# Autodesk Inventor assembly: Team_2374
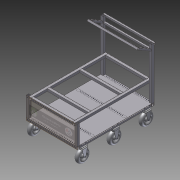
[picture p0: Inventor's stored thumbnail of the model, 180x180]
Saved by Autodesk Inventor 2012 (Build 160160000, 160)
## iProperties
Created: 2011-10-19
Part Number: Team_2374
Document SubType Name: Assembly
Designer: Ian Walters
Mass: 25411.4 g
Surface Area: 59424.9 cm^2
Volume: 9376.89 cm^3
Density: 2.71 g/cm^3
_SolveAssemblyDoc: Frame Generator Solve Assembly
_Version: 15.0.0
Author: Ian Walters
## Documents named in this file (32)
- C:\Users\robotics\Dropbox\CAD Inventor\Preseason Projects\Cart Competition Cart\Team 2374\Team_2374.iam
- C:\Users\robotics\Dropbox\CAD Inventor\Preseason Projects\Cart Competition Cart\Team 2374\Cart Skeleton.ipt
- C:\Users\robotics\Dropbox\CAD Inventor\Preseason Projects\Cart Competition Cart\Team 2374\Team_2374\Frame\Cart Frame.iam
- C:\Users\robotics\Dropbox\CAD Inventor\Preseason Projects\Cart Competition Cart\Team 2374\Bottom Sheet.ipt
- C:\Users\robotics\Dropbox\CAD Inventor\Preseason Projects\Cart Competition Cart\Team 2374\IFI 114 - .1875 x 0.25.ipt
- C:\Users\robotics\Dropbox\CAD Inventor\Preseason Projects\Cart Competition Cart\Team 2374\Fixed Caster.iam
- C:\Users\robotics\Dropbox\CAD Inventor\Preseason Projects\Cart Competition Cart\Team 2374\Team_2374\Design Accelerator\Bolted Connection1.iam
- C:\Users\robotics\Dropbox\CAD Inventor\Preseason Projects\Cart Competition Cart\Team 2374\Team_2374\Design Accelerator\Bolted Connection2.iam
- C:\Users\robotics\Dropbox\CAD Inventor\Preseason Projects\Cart Competition Cart\Team 2374\Team_2374\Design Accelerator\Bolted Connection3.iam
- C:\Users\robotics\Dropbox\CAD Inventor\Preseason Projects\Cart Competition Cart\Team 2374\Team_2374\Design Accelerator\Bolted Connection4.iam
- C:\Users\robotics\Dropbox\CAD Inventor\Preseason Projects\Cart Competition Cart\Team 2374\Team_2374\Design Accelerator\Bolted Connection5.iam
- C:\Users\robotics\Dropbox\CAD Inventor\Preseason Projects\Cart Competition Cart\Team 2374\Team_2374\Design Accelerator\Bolted Connection6.iam
- C:\Users\robotics\Dropbox\CAD Inventor\Preseason Projects\Cart Competition Cart\Team 2374\Team_2374\Design Accelerator\Bolted Connection7.iam
- C:\Users\robotics\Dropbox\CAD Inventor\Preseason Projects\Cart Competition Cart\Team 2374\Team_2374\Design Accelerator\Bolted Connection8.iam
- C:\Users\robotics\Dropbox\CAD Inventor\Preseason Projects\Cart Competition Cart\Team 2374\Front Screen.ipt
- C:\Users\robotics\Dropbox\CAD Inventor\Preseason Projects\Cart Competition Cart\Team 2374\Rotation Caster.iam
- C:\Users\robotics\Dropbox\CAD Inventor\Preseason Projects\Cart Competition Cart\Team 2374\Team_2374\Design Accelerator\Bolted Connection9.iam
- C:\Users\robotics\Dropbox\CAD Inventor\Preseason Projects\Cart Competition Cart\Team 2374\Team_2374\Design Accelerator\Bolted Connection10.iam
- C:\Users\robotics\Dropbox\CAD Inventor\Preseason Projects\Cart Competition Cart\Team 2374\Team_2374\Design Accelerator\Bolted Connection11.iam
- C:\Users\robotics\Dropbox\CAD Inventor\Preseason Projects\Cart Competition Cart\Team 2374\Team_2374\Design Accelerator\Bolted Connection12.iam
- C:\Users\robotics\Dropbox\CAD Inventor\Preseason Projects\Cart Competition Cart\Team 2374\Team_2374\Design Accelerator\Bolted Connection13.iam
- C:\Users\robotics\Dropbox\CAD Inventor\Preseason Projects\Cart Competition Cart\Team 2374\Team_2374\Design Accelerator\Bolted Connection14.iam
- C:\Users\robotics\Dropbox\CAD Inventor\Preseason Projects\Cart Competition Cart\Team 2374\Team_2374\Design Accelerator\Bolted Connection15.iam
- C:\Users\robotics\Dropbox\CAD Inventor\Preseason Projects\Cart Competition Cart\Team 2374\Team_2374\Design Accelerator\Bolted Connection16.iam
- C:\Users\robotics\Dropbox\CAD Inventor\Preseason Projects\Cart Competition Cart\Team 2374\Team_2374\Design Accelerator\Bolted Connection17.iam
- C:\Users\robotics\Dropbox\CAD Inventor\Preseason Projects\Cart Competition Cart\Team 2374\Team_2374\Design Accelerator\Bolted Connection18.iam
- C:\Users\robotics\Dropbox\CAD Inventor\Preseason Projects\Cart Competition Cart\Team 2374\Team_2374\Design Accelerator\Bolted Connection19.iam
- C:\Users\robotics\Dropbox\CAD Inventor\Preseason Projects\Cart Competition Cart\Team 2374\Team_2374\Design Accelerator\Bolted Connection20.iam
- C:\Users\robotics\Dropbox\CAD Inventor\Preseason Projects\Cart Competition Cart\Team 2374\Team_2374\Design Accelerator\Bolted Connection21.iam
- C:\Users\robotics\Dropbox\CAD Inventor\Preseason Projects\Cart Competition Cart\Team 2374\Team_2374\Design Accelerator\Bolted Connection22.iam
- C:\Users\robotics\Dropbox\CAD Inventor\Preseason Projects\Cart Competition Cart\Team 2374\Team_2374\Design Accelerator\Bolted Connection23.iam
- C:\Users\robotics\Dropbox\CAD Inventor\Preseason Projects\Cart Competition Cart\Team 2374\Team_2374\Design Accelerator\Bolted Connection24.iam
## Components (200 placed, 8 different names)
1. Cart Skeleton:1
2. Cart Frame:1 [sub-assembly] — Mate:1, Mate:2, Mate:3, Mate:4, Mate:5, Flush:1, Flush:2, Mate:26, Insert:11, Insert:12, Mate:29, Mate:30, Mate:31, Mate:32, Mate:33, Mate:34, Mate:35, Mate:36, Mate:37, Mate:38, Mate:39, Mate:40, Mate:41, Mate:42, Mate:43, Mate:44, Mate:45, Insert:13, Mate:46, Insert:14, Mate:47, Insert:15, Mate:48, Insert:16, Mate:49, Mate:50, Mate:51, Mate:52, Mate:53, Mate:54, Mate:55, Mate:56, Mate:57, Mate:58, Mate:59, Mate:60, Mate:61, Mate:62, Mate:63, Mate:64, Mate:65, Mate:66, Mate:67, Mate:68, Mate:69, Mate:70, Mate:71, Mate:72, Mate:73, Mate:74, Mate:75, Mate:76, Mate:77, Mate:78, Mate:79, Mate:80
3. Bottom Sheet:1 — Mate:1, Mate:2, Mate:3, Insert:1, Insert:2, Insert:3, Insert:4
4. Fixed Caster:1 [sub-assembly] — Mate:5, Insert:11
5. Fixed Caster:2 [sub-assembly] — Mate:4, Insert:12
6. Bolted Connection:1 [sub-assembly] — Mate:43, Mate:44
7. Bolted Connection:2 [sub-assembly] — Mate:29, Mate:30
8. Bolted Connection:3 [sub-assembly] — Mate:31, Mate:32
9. Bolted Connection:4 [sub-assembly] — Mate:33, Mate:34
10. Bolted Connection:5 [sub-assembly] — Mate:35, Mate:36
11. Bolted Connection:6 [sub-assembly] — Mate:37, Mate:38
12. Bolted Connection:7 [sub-assembly] — Mate:39, Mate:40
13. Bolted Connection:8 [sub-assembly] — Mate:41, Mate:42
14. Front Screen:1 — Flush:1, Flush:2, Mate:26, Insert:7, Insert:8, Insert:9, Insert:10
15. IFI 114 - .1875 x 0.25:109 — Insert:7
16. IFI 114 - .1875 x 0.25:142 — Insert:10
17. Rotation Caster:1 [sub-assembly] — Mate:45, Insert:13
18. Rotation Caster:2 [sub-assembly] — Mate:46, Insert:14
19. Rotation Caster:3 [sub-assembly] — Mate:47, Insert:15
20. Rotation Caster:4 [sub-assembly] — Mate:48, Insert:16
21. Bolted Connection:9 [sub-assembly] — Mate:49, Mate:50
22. Bolted Connection:10 [sub-assembly] — Mate:51, Mate:52
23. Bolted Connection:11 [sub-assembly] — Mate:53, Mate:54
24. Bolted Connection:12 [sub-assembly] — Mate:55, Mate:56
25. Bolted Connection:13 [sub-assembly] — Mate:57, Mate:58
26. Bolted Connection:14 [sub-assembly] — Mate:59, Mate:60
27. Bolted Connection:15 [sub-assembly] — Mate:61, Mate:62
28. Bolted Connection:16 [sub-assembly] — Mate:63, Mate:64
29. Bolted Connection:17 [sub-assembly] — Mate:65, Mate:66
30. Bolted Connection:18 [sub-assembly] — Mate:67, Mate:68
31. Bolted Connection:19 [sub-assembly] — Mate:69, Mate:70
32. Bolted Connection:20 [sub-assembly] — Mate:71, Mate:72
33. Bolted Connection:21 [sub-assembly] — Mate:73, Mate:74
34. Bolted Connection:22 [sub-assembly] — Mate:75, Mate:76
35. Bolted Connection:23 [sub-assembly] — Mate:77, Mate:78
36. Bolted Connection:24 [sub-assembly] — Mate:79, Mate:80
37. IFI 114 - .1875 x 0.25:1 — Insert:1
38. IFI 114 - .1875 x 0.25:2 — Insert:2
39. IFI 114 - .1875 x 0.25:3 — Insert:3
40. IFI 114 - .1875 x 0.25:4 — Insert:4
41. IFI 114 - .1875 x 0.25:5
42. IFI 114 - .1875 x 0.25:6
43. IFI 114 - .1875 x 0.25:7
44. IFI 114 - .1875 x 0.25:8
45. IFI 114 - .1875 x 0.25:9
46. IFI 114 - .1875 x 0.25:10
47. IFI 114 - .1875 x 0.25:11
48. IFI 114 - .1875 x 0.25:12
49. IFI 114 - .1875 x 0.25:13
50. IFI 114 - .1875 x 0.25:14
51. IFI 114 - .1875 x 0.25:15
52. IFI 114 - .1875 x 0.25:16
53. IFI 114 - .1875 x 0.25:17
54. IFI 114 - .1875 x 0.25:18
55. IFI 114 - .1875 x 0.25:19
56. IFI 114 - .1875 x 0.25:20
57. IFI 114 - .1875 x 0.25:21
58. IFI 114 - .1875 x 0.25:22
59. IFI 114 - .1875 x 0.25:23
60. IFI 114 - .1875 x 0.25:24
61. IFI 114 - .1875 x 0.25:25
62. IFI 114 - .1875 x 0.25:26
63. IFI 114 - .1875 x 0.25:27
64. IFI 114 - .1875 x 0.25:28
65. IFI 114 - .1875 x 0.25:29
66. IFI 114 - .1875 x 0.25:30
67. IFI 114 - .1875 x 0.25:31
68. IFI 114 - .1875 x 0.25:32
69. IFI 114 - .1875 x 0.25:33
70. IFI 114 - .1875 x 0.25:34
71. IFI 114 - .1875 x 0.25:35
72. IFI 114 - .1875 x 0.25:36
73. IFI 114 - .1875 x 0.25:37
74. IFI 114 - .1875 x 0.25:38
75. IFI 114 - .1875 x 0.25:39
76. IFI 114 - .1875 x 0.25:40
77. IFI 114 - .1875 x 0.25:41
78. IFI 114 - .1875 x 0.25:42
79. IFI 114 - .1875 x 0.25:43
80. IFI 114 - .1875 x 0.25:44
81. IFI 114 - .1875 x 0.25:45
82. IFI 114 - .1875 x 0.25:46
83. IFI 114 - .1875 x 0.25:47
84. IFI 114 - .1875 x 0.25:48
85. IFI 114 - .1875 x 0.25:49
86. IFI 114 - .1875 x 0.25:50
87. IFI 114 - .1875 x 0.25:51
88. IFI 114 - .1875 x 0.25:52
89. IFI 114 - .1875 x 0.25:53
90. IFI 114 - .1875 x 0.25:54
91. IFI 114 - .1875 x 0.25:55
92. IFI 114 - .1875 x 0.25:56
93. IFI 114 - .1875 x 0.25:57
94. IFI 114 - .1875 x 0.25:58
95. IFI 114 - .1875 x 0.25:59
96. IFI 114 - .1875 x 0.25:60
97. IFI 114 - .1875 x 0.25:61
98. IFI 114 - .1875 x 0.25:62
99. IFI 114 - .1875 x 0.25:63
100. IFI 114 - .1875 x 0.25:64
101. IFI 114 - .1875 x 0.25:65
102. IFI 114 - .1875 x 0.25:66
103. IFI 114 - .1875 x 0.25:67
104. IFI 114 - .1875 x 0.25:68
105. IFI 114 - .1875 x 0.25:69
106. IFI 114 - .1875 x 0.25:70
107. IFI 114 - .1875 x 0.25:71
108. IFI 114 - .1875 x 0.25:72
109. IFI 114 - .1875 x 0.25:73
110. IFI 114 - .1875 x 0.25:74
111. IFI 114 - .1875 x 0.25:75
112. IFI 114 - .1875 x 0.25:76
113. IFI 114 - .1875 x 0.25:77
114. IFI 114 - .1875 x 0.25:78
115. IFI 114 - .1875 x 0.25:79
116. IFI 114 - .1875 x 0.25:80
117. IFI 114 - .1875 x 0.25:81
118. IFI 114 - .1875 x 0.25:82
119. IFI 114 - .1875 x 0.25:83
120. IFI 114 - .1875 x 0.25:84
121. IFI 114 - .1875 x 0.25:85
122. IFI 114 - .1875 x 0.25:86
123. IFI 114 - .1875 x 0.25:87
124. IFI 114 - .1875 x 0.25:88
125. IFI 114 - .1875 x 0.25:89
126. IFI 114 - .1875 x 0.25:90
127. IFI 114 - .1875 x 0.25:91
128. IFI 114 - .1875 x 0.25:92
129. IFI 114 - .1875 x 0.25:93
130. IFI 114 - .1875 x 0.25:94
131. IFI 114 - .1875 x 0.25:95
132. IFI 114 - .1875 x 0.25:96
133. IFI 114 - .1875 x 0.25:97
134. IFI 114 - .1875 x 0.25:98
135. IFI 114 - .1875 x 0.25:99
136. IFI 114 - .1875 x 0.25:100
137. IFI 114 - .1875 x 0.25:101
138. IFI 114 - .1875 x 0.25:102
139. IFI 114 - .1875 x 0.25:103
140. IFI 114 - .1875 x 0.25:104
141. IFI 114 - .1875 x 0.25:105
142. IFI 114 - .1875 x 0.25:106
143. IFI 114 - .1875 x 0.25:107
144. IFI 114 - .1875 x 0.25:108
145. IFI 114 - .1875 x 0.25:110 — Insert:8
146. IFI 114 - .1875 x 0.25:111
147. IFI 114 - .1875 x 0.25:112
148. IFI 114 - .1875 x 0.25:113
149. IFI 114 - .1875 x 0.25:114
150. IFI 114 - .1875 x 0.25:115
151. IFI 114 - .1875 x 0.25:116
152. IFI 114 - .1875 x 0.25:117
153. IFI 114 - .1875 x 0.25:118
154. IFI 114 - .1875 x 0.25:119
155. IFI 114 - .1875 x 0.25:120
156. IFI 114 - .1875 x 0.25:121
157. IFI 114 - .1875 x 0.25:122
158. IFI 114 - .1875 x 0.25:123
159. IFI 114 - .1875 x 0.25:124
160. IFI 114 - .1875 x 0.25:125
161. IFI 114 - .1875 x 0.25:126
162. IFI 114 - .1875 x 0.25:127
163. IFI 114 - .1875 x 0.25:128
164. IFI 114 - .1875 x 0.25:129
165. IFI 114 - .1875 x 0.25:130
166. IFI 114 - .1875 x 0.25:131
167. IFI 114 - .1875 x 0.25:132
168. IFI 114 - .1875 x 0.25:133
169. IFI 114 - .1875 x 0.25:134
170. IFI 114 - .1875 x 0.25:135
171. IFI 114 - .1875 x 0.25:136
172. IFI 114 - .1875 x 0.25:137
173. IFI 114 - .1875 x 0.25:138
174. IFI 114 - .1875 x 0.25:139
175. IFI 114 - .1875 x 0.25:140
176. IFI 114 - .1875 x 0.25:141 — Insert:9
177. IFI 114 - .1875 x 0.25:143
178. IFI 114 - .1875 x 0.25:144
179. IFI 114 - .1875 x 0.25:145
180. IFI 114 - .1875 x 0.25:146
181. IFI 114 - .1875 x 0.25:147
182. IFI 114 - .1875 x 0.25:148
183. IFI 114 - .1875 x 0.25:149
184. IFI 114 - .1875 x 0.25:150
185. IFI 114 - .1875 x 0.25:151
186. IFI 114 - .1875 x 0.25:152
187. IFI 114 - .1875 x 0.25:153
188. IFI 114 - .1875 x 0.25:154
189. IFI 114 - .1875 x 0.25:155
190. IFI 114 - .1875 x 0.25:156
191. IFI 114 - .1875 x 0.25:157
192. IFI 114 - .1875 x 0.25:158
193. IFI 114 - .1875 x 0.25:159
194. IFI 114 - .1875 x 0.25:160
195. IFI 114 - .1875 x 0.25:161
196. IFI 114 - .1875 x 0.25:162
197. IFI 114 - .1875 x 0.25:163
198. IFI 114 - .1875 x 0.25:164
199. IFI 114 - .1875 x 0.25:165
200. IFI 114 - .1875 x 0.25:166
## Component patterns: (27 elements, first: IFI 114 - .1875 x 0.25:1 + IFI 114 - .1875 x 0.25:2 + IFI 114 - .1875 x 0.25:3 + IFI 114 - .1875 x 0.25:4), (31 elements, first: IFI 114 - .1875 x 0.25:110), (25 elements, first: IFI 114 - .1875 x 0.25:141)
## Relationships (74: Mate 58, Insert 14, Flush 2)
- Mate:1: Cart Frame:1 ↔ Bottom Sheet:1
- Mate:2: Cart Frame:1 ↔ Bottom Sheet:1
- Mate:3: Cart Frame:1 ↔ Bottom Sheet:1
- Insert:1: Bottom Sheet:1 ↔ IFI 114 - .1875 x 0.25:1
- Insert:2: Bottom Sheet:1 ↔ IFI 114 - .1875 x 0.25:2
- Insert:3: Bottom Sheet:1 ↔ IFI 114 - .1875 x 0.25:3
- Insert:4: Bottom Sheet:1 ↔ IFI 114 - .1875 x 0.25:4
- Mate:4: Cart Frame:1 ↔ Fixed Caster:2
- Mate:5: Cart Frame:1 ↔ Fixed Caster:1
- Flush:1: Cart Frame:1 ↔ Front Screen:1
- Flush:2: Cart Frame:1 ↔ Front Screen:1
- Mate:26: Cart Frame:1 ↔ Front Screen:1
- Insert:7: Front Screen:1 ↔ IFI 114 - .1875 x 0.25:109
- Insert:8: Front Screen:1 ↔ IFI 114 - .1875 x 0.25:110
- Insert:9: Front Screen:1 ↔ IFI 114 - .1875 x 0.25:141
- Insert:10: Front Screen:1 ↔ IFI 114 - .1875 x 0.25:142
- Insert:11: Cart Frame:1 ↔ Fixed Caster:1
- Insert:12: Cart Frame:1 ↔ Fixed Caster:2
- Mate:29: Cart Frame:1 ↔ Bolted Connection:2
- Mate:30: Cart Frame:1 ↔ Bolted Connection:2
- Mate:31: Cart Frame:1 ↔ Bolted Connection:3
- Mate:32: Cart Frame:1 ↔ Bolted Connection:3
- Mate:33: Cart Frame:1 ↔ Bolted Connection:4
- Mate:34: Cart Frame:1 ↔ Bolted Connection:4
- Mate:35: Cart Frame:1 ↔ Bolted Connection:5
- Mate:36: Cart Frame:1 ↔ Bolted Connection:5
- Mate:37: Cart Frame:1 ↔ Bolted Connection:6
- Mate:38: Cart Frame:1 ↔ Bolted Connection:6
- Mate:39: Cart Frame:1 ↔ Bolted Connection:7
- Mate:40: Cart Frame:1 ↔ Bolted Connection:7
- Mate:41: Cart Frame:1 ↔ Bolted Connection:8
- Mate:42: Cart Frame:1 ↔ Bolted Connection:8
- Mate:43: Cart Frame:1 ↔ Bolted Connection:1
- Mate:44: Cart Frame:1 ↔ Bolted Connection:1
- Mate:45: Cart Frame:1 ↔ Rotation Caster:1
- Insert:13: Cart Frame:1 ↔ Rotation Caster:1
- Mate:46: Cart Frame:1 ↔ Rotation Caster:2
- Insert:14: Cart Frame:1 ↔ Rotation Caster:2
- Mate:47: Cart Frame:1 ↔ Rotation Caster:3
- Insert:15: Cart Frame:1 ↔ Rotation Caster:3
- Mate:48: Cart Frame:1 ↔ Rotation Caster:4
- Insert:16: Cart Frame:1 ↔ Rotation Caster:4
- Mate:49: Cart Frame:1 ↔ Bolted Connection:9
- Mate:50: Cart Frame:1 ↔ Bolted Connection:9
- Mate:51: Cart Frame:1 ↔ Bolted Connection:10
- Mate:52: Cart Frame:1 ↔ Bolted Connection:10
- Mate:53: Cart Frame:1 ↔ Bolted Connection:11
- Mate:54: Cart Frame:1 ↔ Bolted Connection:11
- Mate:55: Cart Frame:1 ↔ Bolted Connection:12
- Mate:56: Cart Frame:1 ↔ Bolted Connection:12
- Mate:57: Cart Frame:1 ↔ Bolted Connection:13
- Mate:58: Cart Frame:1 ↔ Bolted Connection:13
- Mate:59: Cart Frame:1 ↔ Bolted Connection:14
- Mate:60: Cart Frame:1 ↔ Bolted Connection:14
- Mate:61: Cart Frame:1 ↔ Bolted Connection:15
- Mate:62: Cart Frame:1 ↔ Bolted Connection:15
- Mate:63: Cart Frame:1 ↔ Bolted Connection:16
- Mate:64: Cart Frame:1 ↔ Bolted Connection:16
- Mate:65: Cart Frame:1 ↔ Bolted Connection:17
- Mate:66: Cart Frame:1 ↔ Bolted Connection:17
- Mate:67: Cart Frame:1 ↔ Bolted Connection:18
- Mate:68: Cart Frame:1 ↔ Bolted Connection:18
- Mate:69: Cart Frame:1 ↔ Bolted Connection:19
- Mate:70: Cart Frame:1 ↔ Bolted Connection:19
- Mate:71: Cart Frame:1 ↔ Bolted Connection:20
- Mate:72: Cart Frame:1 ↔ Bolted Connection:20
- Mate:73: Cart Frame:1 ↔ Bolted Connection:21
- Mate:74: Cart Frame:1 ↔ Bolted Connection:21
- Mate:75: Cart Frame:1 ↔ Bolted Connection:22
- Mate:76: Cart Frame:1 ↔ Bolted Connection:22
- Mate:77: Cart Frame:1 ↔ Bolted Connection:23
- Mate:78: Cart Frame:1 ↔ Bolted Connection:23
- Mate:79: Cart Frame:1 ↔ Bolted Connection:24
- Mate:80: Cart Frame:1 ↔ Bolted Connection:24
